# Autodesk Inventor assembly: Photo-Sensor
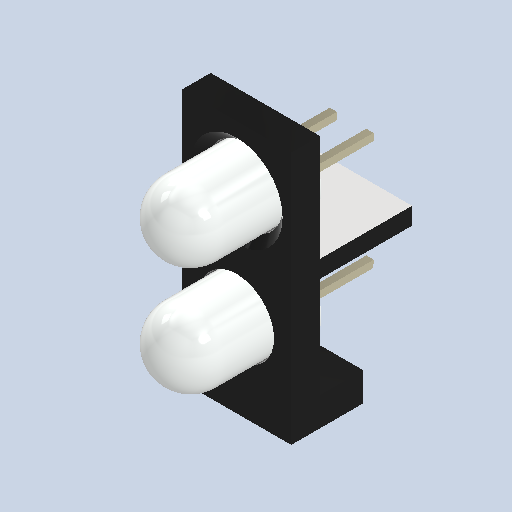
[picture p0: Inventor's stored thumbnail of the model, 512x512]
Saved by Autodesk Inventor 2022 (Build 260153000, 153)
## iProperties
Created: 2024-06-27
Part Number: Photo-Sensor
Document SubType Name: Assembly
Designer: yamashita1
Author: yamashita1
## Documents named in this file (3)
- G:\マイドライブ\project\micro-mouse\3D-Model\Photo-Sensor.iam
- G:\マイドライブ\project\micro-mouse\3D-Model\LED-Spacer1.ipt
- G:\マイドライブ\project\micro-mouse\3D-Model\LED.ipt
## Components (3 placed, 2 different names)
1. LED-Spacer1:1 — メイト:1, メイト:2, メイト:3, メイト:4
2. LED:1 — メイト:1, メイト:3
3. LED:2 — メイト:2, メイト:4
## Relationships (4: Mate 4)
- メイト:1 [Mate]: LED-Spacer1:1 ↔ LED:1
- メイト:2 [Mate]: LED-Spacer1:1 ↔ LED:2
- メイト:3 [Mate]: LED-Spacer1:1 ↔ LED:1
- メイト:4 [Mate]: LED-Spacer1:1 ↔ LED:2
